# Autodesk Inventor assembly: UBG-Electronics
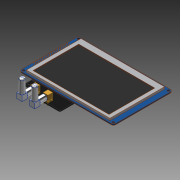
[picture p0: Inventor's stored thumbnail of the model, 180x180]
Saved by Autodesk Inventor 2019.4 (Build 234330000, 330)
## iProperties
Created: 2017-11-11
Part Number: UBG-Electronics
Document SubType Name: Assembly
Designer: rYan
Author: rYan
## Documents named in this file (3)
- D:\TIGERsGIT\Hardware\mechanik\2020\Inventor\Base Station\UBG-Electronics.iam
- D:\TIGERsGIT\Hardware\mechanik\2020\Inventor\Base Station\MG-Base Station PCB.iam
- D:\TIGERsGIT\Hardware\mechanik\2020\Inventor\Purchased Parts\TFT-CP11009.ipt
## Components (2 placed, 2 different names)
1. MG-Base Station v3:1 [sub-assembly] — Passend:1, Fluchtend:1, Fluchtend:2
2. TFT-CP11009:1 — Passend:1, Fluchtend:1, Fluchtend:2
## Relationships (3: Flush 2, Mate 1)
- Passend:1 [Mate]: MG-Base Station v3:1 ↔ TFT-CP11009:1
- Fluchtend:1 [Flush] (-0.0635 mm): MG-Base Station v3:1 ↔ TFT-CP11009:1
- Fluchtend:2 [Flush]: MG-Base Station v3:1 ↔ TFT-CP11009:1
